# Autodesk Inventor assembly: 102
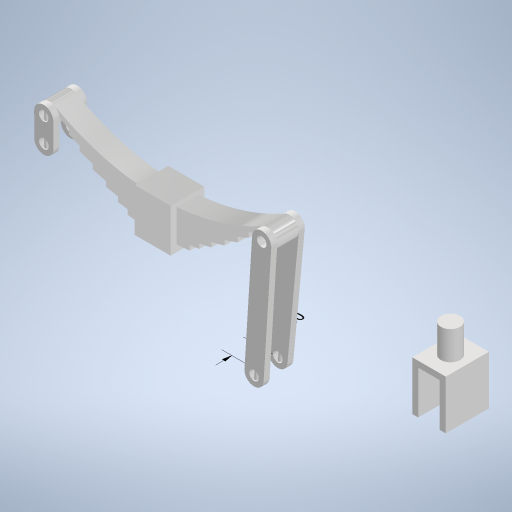
[picture p0: Inventor's stored thumbnail of the model, 512x512]
Saved by Autodesk Inventor 2024.2 (Build 282272000, 272)
## iProperties
Created: 2024-11-02
Part Number: 102
Document SubType Name: Assembly
Designer: Jimena Brenes
Author: Jimena Brenes
## Documents named in this file (5)
- C:\Users\Jimena Brenes\OneDrive\Escritorio\1-102\102.iam
- C:\Users\Jimena Brenes\OneDrive\Escritorio\locomotora\HUDSON 1-14 LEAFSPRING HANGER-1.ipt
- C:\Users\Jimena Brenes\OneDrive\Escritorio\locomotora\HUDSON-1-09-LEAF SPRING PACK.ipt
- C:\Users\Jimena Brenes\OneDrive\Escritorio\locomotora\HUDSON 1-10-LEAFSPRING-AXLE BOX SADDLE.ipt
- C:\Users\Jimena Brenes\OneDrive\Escritorio\locomotora\1-16.ipt
## Components (6 placed, 4 different names)
1. HUDSON 1-14 LEAFSPRING HANGER-1:1 — Mate:3, Mate:4
2. HUDSON 1-14 LEAFSPRING HANGER-1:2 — Mate:1, Mate:2
3. HUDSON-1-09-LEAF SPRING PACK:1 — Mate:1, Mate:2, Mate:3, Mate:4, Mate:5, Mate:6, Mate:7, Mate:8
4. HUDSON 1-10-LEAFSPRING-AXLE BOX SADDLE:1
5. 1-16:1 — Mate:7, Mate:8
6. 1-16:2 — Mate:5, Mate:6
## Relationships (8: Mate 8)
- Mate:1: HUDSON 1-14 LEAFSPRING HANGER-1:2 ↔ HUDSON-1-09-LEAF SPRING PACK:1
- Mate:2: HUDSON 1-14 LEAFSPRING HANGER-1:2 ↔ HUDSON-1-09-LEAF SPRING PACK:1
- Mate:3: HUDSON 1-14 LEAFSPRING HANGER-1:1 ↔ HUDSON-1-09-LEAF SPRING PACK:1
- Mate:4: HUDSON 1-14 LEAFSPRING HANGER-1:1 ↔ HUDSON-1-09-LEAF SPRING PACK:1
- Mate:5: HUDSON-1-09-LEAF SPRING PACK:1 ↔ 1-16:2
- Mate:6: HUDSON-1-09-LEAF SPRING PACK:1 ↔ 1-16:2
- Mate:7: HUDSON-1-09-LEAF SPRING PACK:1 ↔ 1-16:1
- Mate:8: HUDSON-1-09-LEAF SPRING PACK:1 ↔ 1-16:1
